# Autodesk Inventor assembly: Drive
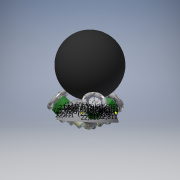
[picture p0: Inventor's stored thumbnail of the model, 180x180]
Saved by Autodesk Inventor 2018.3 (Build 223284000, 284)
## iProperties
Created: 2018-06-30
Part Number: Drive
Material: Generisch
Document SubType Name: Assembly
Designer: JochenAlt
Author: JochenAlt
## Documents named in this file (3)
- D:\Projects\FlowerPot\CAD\Drive.iam
- D:\Projects\FlowerPot\CAD\DriveChain.iam
- D:\Projects\FlowerPot\CAD\Sphere.ipt
## Components (4 placed, 2 different names)
1. Antriebsstrang:1 [sub-assembly] — Passend:1, Fluchtend:2, Passend:3, Passend:6, Passend:7, Passend:10, Passend:12, Passend:13
2. Antriebsstrang:2 [sub-assembly] — Passend:11, Passend:12, Passend:15
3. Antriebsstrang:3 [sub-assembly] — Passend:1, Fluchtend:2, Passend:3, Passend:7, Passend:11, Passend:13, Passend:15
4. Sphere:1 — Passend:10
## Relationships (10: Mate 9, Flush 1)
- Passend:1 [Mate]: Antriebsstrang:1 ↔ Antriebsstrang:3
- Fluchtend:2 [Flush]: Antriebsstrang:1 ↔ Antriebsstrang:3
- Passend:3 [Mate]: Antriebsstrang:1 ↔ Antriebsstrang:3
- Passend:6 [Mate]: Antriebsstrang:1
- Passend:7 [Mate]: Antriebsstrang:1 ↔ Antriebsstrang:3
- Passend:10 [Mate]: Antriebsstrang:1 ↔ Sphere:1
- Passend:11 [Mate]: Antriebsstrang:2 ↔ Antriebsstrang:3
- Passend:12 [Mate]: Antriebsstrang:1 ↔ Antriebsstrang:2
- Passend:13 [Mate]: Antriebsstrang:1 ↔ Antriebsstrang:3
- Passend:15 [Mate]: Antriebsstrang:2 ↔ Antriebsstrang:3
